# Autodesk Inventor assembly: Сборка датчика земли
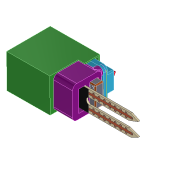
[picture p0: Inventor's stored thumbnail of the model, 180x180]
Saved by Autodesk Inventor 2022 (Build 260153000, 153)
## iProperties
Created: 2023-02-19
Part Number: Сборка датчика земли
Document SubType Name: Assembly
Designer: Egori
Mass: 41.4711 g
Surface Area: 329.412 cm^2
Volume: 41.4711 cm^3
Density: 1 g/cm^3
Author: Egori
## Documents named in this file (6)
- C:\Теплица\Сборка датчика земли.iam
- C:\Теплица\кронштейн для земли.ipt
- C:\Теплица\Soil-Moisture-Sensor-Probe.ipt
- C:\Теплица\сборка мк для земли.iam
- C:\Теплица\крышка земли.ipt
- C:\Теплица\аккумулятор.ipt
## Components (5 placed, 5 different names)
1. кронштейн для земли:1 — Жесткий:1, Совмещение:1, Совмещение:2
2. Soil-Moisture-Sensor-Probe:1 — Жесткий:1
3. сборка мк для земли:1 [sub-assembly] — Совмещение:1, Совмещение:3
4. крышка земли:1 — Совмещение:3
5. аккумулятор:1 — Совмещение:2
## Relationships (4: Mate 3, WeldJoint 1)
- Жесткий:1 [WeldJoint]: кронштейн для земли:1 ↔ Soil-Moisture-Sensor-Probe:1
- Совмещение:1 [Mate]: кронштейн для земли:1 ↔ сборка мк для земли:1
- Совмещение:2 [Mate]: кронштейн для земли:1 ↔ аккумулятор:1
- Совмещение:3 [Mate]: сборка мк для земли:1 ↔ крышка земли:1
